# Autodesk Inventor assembly: Assembly1
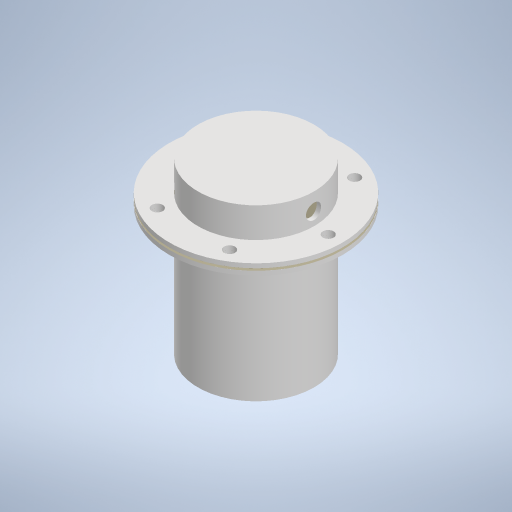
[picture p0: Inventor's stored thumbnail of the model, 512x512]
Saved by Autodesk Inventor 2023 (Build 270158000, 158)
## iProperties
Created: 2023-01-27
Part Number: Assembly1
Document SubType Name: Assembly
Designer: remidm
Author: remidm
## Documents named in this file (5)
- C:\Projects\permeation_rig\design\InnerVessel.iam
- C:\Projects\permeation_rig\design\DownstreamVolume.ipt
- C:\Projects\permeation_rig\design\membrane.ipt
- C:\Projects\permeation_rig\design\salt.ipt
- C:\Projects\permeation_rig\design\UpstreamVolume.ipt
## Components (4 placed, 4 different names)
1. DownstreamVolume:1 — Mate:1, Mate:3, Mate:10, Mate:11, Mate:13, Mate:14, Mate:15
2. membrane:1 — Mate:3, Mate:6, Mate:9, Mate:12, Mate:13
3. salt:1 — Mate:1, Mate:9
4. UpstreamVolume:1 — Mate:6, Mate:10, Mate:11, Mate:12, Flush:1
## Relationships (11: Mate 10, Flush 1)
- Mate:1: DownstreamVolume:1 ↔ salt:1
- Mate:3: DownstreamVolume:1 ↔ membrane:1
- Mate:6: membrane:1 ↔ UpstreamVolume:1
- Mate:9: membrane:1 ↔ salt:1
- Mate:10: DownstreamVolume:1 ↔ UpstreamVolume:1
- Mate:11: DownstreamVolume:1 ↔ UpstreamVolume:1
- Mate:12: membrane:1 ↔ UpstreamVolume:1
- Mate:13: DownstreamVolume:1 ↔ membrane:1
- Mate:14: DownstreamVolume:1
- Mate:15: DownstreamVolume:1
- Flush:1: UpstreamVolume:1
